# Autodesk Inventor assembly: shin_assembly
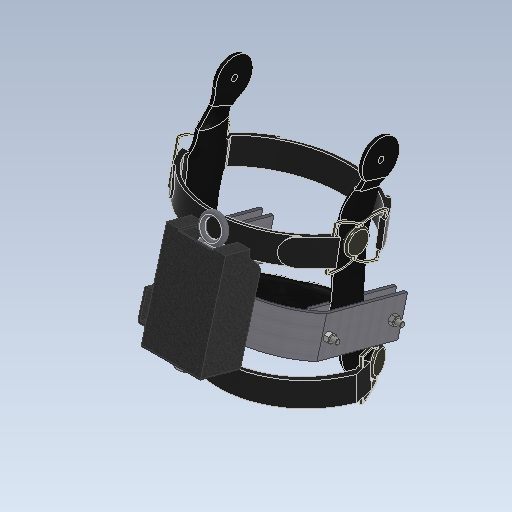
[picture p0: Inventor's stored thumbnail of the model, 512x512]
Saved by Autodesk Inventor 2025.2 (Build 292293000, 293)
## iProperties
Created: 2025-02-17
Part Number: shin_assembly
Document SubType Name: Assembly
Designer: email
Author: email
## Documents named in this file (7)
- C:\Users\email\Desktop\Projects\Capstone\4TB6\CAD_Model\thigh_mount_2\shin_assembly.iam
- C:\Users\email\Desktop\Projects\Capstone\4TB6\CAD_Model\thigh_mount_2\shin.ipt
- C:\Users\email\Desktop\Projects\Capstone\4TB6\CAD_Model\thigh_mount_2\shin_bracket_assem.iam
- C:\Users\email\Desktop\Projects\Capstone\4TB6\CAD_Model\thigh_mount_2\brace_tabs.ipt
- C:\Users\email\Desktop\Projects\Capstone\4TB6\CAD_Model\thigh_mount_2\brace_tabs_half.ipt
- C:\Users\email\Desktop\Projects\Capstone\4TB6\CAD_Model\thigh_mount_2\thigh_strap_04.ipt
- C:\Users\email\Desktop\Projects\Capstone\4TB6\CAD_Model\thigh_mount_2\thigh_strap_05.ipt
## Components (8 placed, 6 different names)
1. shin:1 — Flush:2, Mate:1, Angle:1, Mate:2, Mate:3, Angle:5, Mate:4, Mate:5, Angle:6, Mate:6, Mate:7, Mate:8, Mate:9, Mate:10, Mate:11
2. shin_bracket_assem:1 [sub-assembly] — Flush:2, Mate:1, Angle:1, Mate:2, Mate:3
3. brace_tabs:1 — Angle:6, Mate:6, Mate:7
4. brace_tabs:2 — Angle:5, Mate:4, Mate:5
5. brace_tabs_half:1 — Mate:10, Mate:11
6. brace_tabs_half:2 — Mate:8, Mate:9
7. thigh_strap_04:1
8. thigh_strap_05:1
## Relationships (15: Mate 11, Angle 3, Flush 1)
- Flush:2 (-120 mm): shin:1 ↔ shin_bracket_assem:1
- Mate:1 (50 mm): shin:1 ↔ shin_bracket_assem:1
- Angle:1 (15 deg): shin:1 ↔ shin_bracket_assem:1
- Mate:2: shin:1 ↔ shin_bracket_assem:1
- Mate:3 (120 mm): shin:1 ↔ shin_bracket_assem:1
- Angle:5 (230 deg): shin:1 ↔ brace_tabs:2
- Mate:4: shin:1 ↔ brace_tabs:2
- Mate:5: shin:1 ↔ brace_tabs:2
- Angle:6 (-10 deg): shin:1 ↔ brace_tabs:1
- Mate:6: shin:1 ↔ brace_tabs:1
- Mate:7: shin:1 ↔ brace_tabs:1
- Mate:8: shin:1 ↔ brace_tabs_half:2
- Mate:9: shin:1 ↔ brace_tabs_half:2
- Mate:10: shin:1 ↔ brace_tabs_half:1
- Mate:11 (3 mm): shin:1 ↔ brace_tabs_half:1
